# Autodesk Inventor assembly: XT661-4C-X427
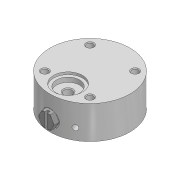
[picture p0: Inventor's stored thumbnail of the model, 180x180]
Saved by Autodesk Inventor 2021 (Build 250183000, 183)
## iProperties
Company: CADENAS
Created: 2021-04-06
Part Number: XT661-4C-X427
Description: STEP AP214
Document SubType Name: Assembly
Designer: romanp
Sending System: PARTsolutions
Title: p:/temp/worker_40/temp/exporttempdir_1948_29_VMMRn/format_0/XT661-4C-X427.stp
Author: License CC BY-ND 4.0
Revision Number: NONE
## Documents named in this file (4)
- C:\Users\romanp\Desktop\Gripper_Project\Gripper_Parts\Cyclone_New\Cyclone\XT661-4C-X427.iam
- C:\Users\romanp\Desktop\Gripper_Project\Gripper_Parts\Cyclone_New\Cyclone\_XT661-4C-X427_DUMMY.ipt
- C:\Users\romanp\Desktop\Gripper_Project\Gripper_Parts\Cyclone_New\Cyclone\_XT661-4C-X427_BODY.ipt
- C:\Users\romanp\Desktop\Gripper_Project\Gripper_Parts\Cyclone_New\Cyclone\_M-5P.ipt
## Components (4 placed, 4 different names)
1. NAUO1
2. NAUO2 — Insert:1
3. NAUO4
4. _M-5P:3 — Insert:1
## Relationships (1: Insert 1)
- Insert:1: NAUO2 ↔ _M-5P:3
